# Autodesk Inventor assembly: Сборка2
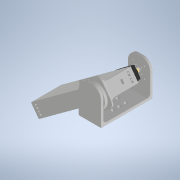
[picture p0: Inventor's stored thumbnail of the model, 180x180]
Saved by Autodesk Inventor 2022 (Build 260153000, 153)
## iProperties
Created: 2023-02-27
Part Number: Сборка2
Document SubType Name: Assembly
Designer: Pavel
Author: Pavel
## Documents named in this file (5)
- G:\Новая папка\Сборка2.iam
- G:\Новая папка\мотор_плеча_2.1-локтя_1_v2.ipt
- G:\Новая папка\servoDS3115mg.iam
- G:\Новая папка\подш.ipt
- G:\Новая папка\мотор_плеча_2_v2.ipt
## Components (4 placed, 4 different names)
1. мотор_плеча_2.1-локтя_1_v2:1 — Совмещение:1, Совмещение:2, Совмещение:3, Совмещение:4, Совмещение:5
2. servoDS3115mg:1 [sub-assembly] — Совмещение:1, Совмещение:2, Совмещение:3, Совмещение:8
3. подш:1 — Совмещение:4, Совмещение:5, Совмещение:6, Совмещение:7
4. мотор_плеча_2_v2:1 — Совмещение:6, Совмещение:7, Совмещение:8
## Relationships (8: Mate 8)
- Совмещение:1 [Mate]: мотор_плеча_2.1-локтя_1_v2:1 ↔ servoDS3115mg:1
- Совмещение:2 [Mate]: мотор_плеча_2.1-локтя_1_v2:1 ↔ servoDS3115mg:1
- Совмещение:3 [Mate]: мотор_плеча_2.1-локтя_1_v2:1 ↔ servoDS3115mg:1
- Совмещение:4 [Mate]: мотор_плеча_2.1-локтя_1_v2:1 ↔ подш:1
- Совмещение:5 [Mate]: мотор_плеча_2.1-локтя_1_v2:1 ↔ подш:1
- Совмещение:6 [Mate]: подш:1 ↔ мотор_плеча_2_v2:1
- Совмещение:7 [Mate]: подш:1 ↔ мотор_плеча_2_v2:1
- Совмещение:8 [Mate] (2 mm): servoDS3115mg:1 ↔ мотор_плеча_2_v2:1
